# Autodesk Inventor assembly: ExternalMoldAssembly
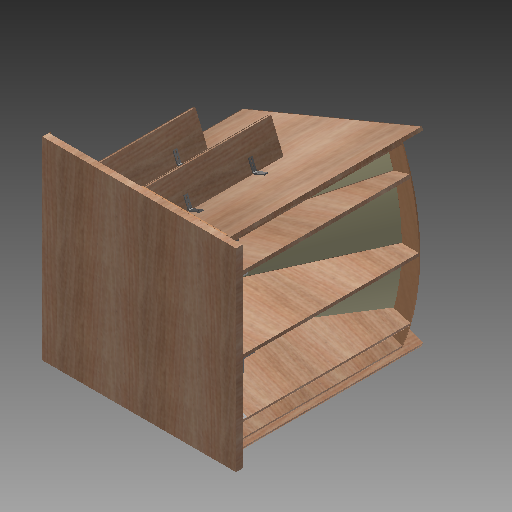
[picture p0: Inventor's stored thumbnail of the model, 512x512]
Saved by Autodesk Inventor 2019 (Build 230136000, 136)
## iProperties
Company: FABLAB Torino
Created: 2019-01-11
Part Number: ExternalMoldAssembly
Document SubType Name: Assembly
Designer: Giancarlo
Project: La Panca - Flower Vase
Mass: 72304.3 g
Surface Area: 89186 cm^2
Volume: 48627 cm^3
Density: 1.48692 g/cm^3
Author: Giancarlo
Title: La Panca - Flower Vase
Subject: Construction MOld
## Documents named in this file (14)
- D:\Giancarlo Bacchio\Documenti\00 - Progetti\30-Inventor\flower vase\ExternalMoldAssembly.iam
- D:\Giancarlo Bacchio\Documenti\00 - Progetti\30-Inventor\flower vase\externalMold_parts\front panel.ipt
- D:\Giancarlo Bacchio\Documenti\00 - Progetti\30-Inventor\flower vase\externalMold_parts\rear panel.ipt
- D:\Giancarlo Bacchio\Documenti\00 - Progetti\30-Inventor\flower vase\externalMold_parts\base1.ipt
- D:\Giancarlo Bacchio\Documenti\00 - Progetti\30-Inventor\flower vase\externalMold_parts\ref1.ipt
- D:\Giancarlo Bacchio\Documenti\00 - Progetti\30-Inventor\flower vase\externalMold_parts\support1.ipt
- D:\Giancarlo Bacchio\Documenti\00 - Progetti\30-Inventor\flower vase\externalMold_parts\frontformer.ipt
- D:\Giancarlo Bacchio\Documenti\00 - Progetti\30-Inventor\flower vase\externalMold_parts\verticalff.ipt
- D:\Giancarlo Bacchio\Documenti\00 - Progetti\30-Inventor\flower vase\externalMold_parts\verticalff1.ipt
- D:\Giancarlo Bacchio\Documenti\00 - Progetti\30-Inventor\flower vase\externalMold_parts\ref3.ipt
- D:\Giancarlo Bacchio\Documenti\00 - Progetti\30-Inventor\flower vase\externalMold_parts\base.ipt
- D:\Giancarlo Bacchio\Documenti\00 - Progetti\30-Inventor\flower vase\externalMold_parts\externalSupportRear1.ipt
- D:\Giancarlo Bacchio\Documenti\00 - Progetti\30-Inventor\flower vase\externalMold_parts\externalSupportRear3.ipt
- D:\Giancarlo Bacchio\Documenti\00 - Progetti\30-Inventor\flower vase\externalMold_parts\JIS G 3350C - 3075     40x40-12.ipt
## Components (53 placed, 13 different names)
1. externalSupportRear3:1 — Flush:19, Flush:20, Mate:86, Mate:88, Mate:90, Mate:92, Mate:94
2. externalSupportRear1:1 — Flush:17, Flush:18
3. externalSupportBase:1 — Flush:19, Flush:20, Mate:76, Mate:78, Mate:80, Mate:82, Mate:84, Mate:106, Flush:26, Mate:120, Mate:125, Flush:27, Mate:126, Mate:128, Mate:130, Mate:132, Mate:133
4. JIS G 3350C - 3075     40x40-12:22 — Mate:133, Mate:135, Flush:31
5. JIS G 3350C - 3075     40x40-12:21 — Mate:132, Mate:137, Flush:32
6. JIS G 3350C - 3075     40x40-12:20 — Mate:128, Mate:136, Flush:33
7. JIS G 3350C - 3075     40x40-12:19 — Mate:126, Mate:127, Flush:28
8. JIS G 3350C - 3075     40x40-12:18 — Mate:116, Mate:117, Mate:118
9. JIS G 3350C - 3075     40x40-12:17 — Mate:114, Mate:115, Mate:124
10. JIS G 3350C - 3075     40x40-12:16 — Mate:112, Mate:113, Mate:123
11. JIS G 3350C - 3075     40x40-12:15 — Mate:110, Mate:111, Mate:119
12. ref1:2 — Mate:106, Mate:107, Flush:26, Mate:108, Mate:109
13. JIS G 3350C - 3075     40x40-12:14 — Mate:103, Mate:104, Mate:109
14. JIS G 3350C - 3075     40x40-12:13 — Mate:102, Mate:105, Mate:108
15. JIS G 3350C - 3075     40x40-12:12 — Mate:99, Mate:100, Mate:101
16. JIS G 3350C - 3075     40x40-12:11 — Mate:88, Mate:89
17. JIS G 3350C - 3075     40x40-12:10 — Mate:94, Mate:95
18. JIS G 3350C - 3075     40x40-12:9 — Mate:96, Mate:97, Mate:98
19. JIS G 3350C - 3075     40x40-12:8 — Mate:92, Mate:93
20. JIS G 3350C - 3075     40x40-12:7 — Mate:90, Mate:91
21. JIS G 3350C - 3075     40x40-12:6 — Mate:86, Mate:87
22. JIS G 3350C - 3075     40x40-12:5 — Mate:84, Mate:85, Flush:25
23. JIS G 3350C - 3075     40x40-12:4 — Mate:82, Mate:83, Flush:24
24. JIS G 3350C - 3075     40x40-12:3 — Mate:80, Mate:81, Flush:23
25. JIS G 3350C - 3075     40x40-12:2 — Mate:78, Mate:79, Flush:22
26. JIS G 3350C - 3075     40x40-12:1 — Mate:76, Mate:77, Flush:21
27. base1:2 — Mate:75, Mate:97, Mate:100, Mate:104, Mate:105
28. base1:3 — Mate:73, Mate:111, Mate:113, Mate:115, Mate:117, Mate:122, Mate:131
29. ref3:1 — Mate:73, Mate:121, Mate:123, Mate:124, Mate:125, Flush:27
30. ref3:2 — Mate:61, Mate:75, Mate:98, Mate:101
31. verticalff1:1 — Mate:81, Flush:23, Mate:91
32. verticalff1:2 — Mate:79, Flush:22, Mate:95
33. verticalff1:3 — Mate:85, Flush:25, Mate:89
34. verticalff1:4 — Flush:17, Flush:18, Mate:77, Flush:21, Mate:93
35. verticalff1:5 — Mate:83, Flush:24, Mate:87
36. frontformer:1 — Flush:10, Flush:11, Flush:12, Mate:17, Flush:13, Mate:19
37. verticalff:1 — Flush:10, Flush:11, Flush:14, Mate:20, Mate:21, Mate:22, Mate:23, Mate:24
38. verticalff:2 — Flush:12, Mate:17
39. verticalff:3 — Flush:13, Mate:19, Mate:25, Mate:26, Mate:27, Mate:28, Mate:29, Mate:30, Mate:31, Mate:32, Mate:33, Mate:34, Mate:35, Mate:36, Mate:37, Mate:38, Mate:39, Mate:40
40. frontformer:2 — Flush:14, Mate:20, Mate:21, Mate:22
41. frontformer:3 — Mate:23, Mate:24, Mate:25
42. frontformer:4 — Mate:26, Mate:27, Mate:28
43. frontformer:5 — Mate:29, Mate:30, Mate:31
44. frontformer:6 — Mate:32, Mate:33, Mate:34
45. frontformer:7 — Mate:38, Mate:39, Mate:40
46. frontformer:8 — Mate:35, Mate:36, Mate:37
47. ref1:1 — Mate:12, Mate:118, Mate:119
48. support1:1 — Mate:112, Mate:114, Mate:120, Mate:121, Mate:122, Mate:135, Flush:31
49. support1:2 — Mate:12, Mate:110, Mate:116, Mate:127, Mate:130, Mate:131, Flush:28
50. support1:3 — Mate:102, Mate:103, Mate:107, Mate:136, Flush:33
51. support1:4 — Mate:61, Mate:96, Mate:99, Mate:137, Flush:32
52. front panel:1
53. rear panel:1
## Relationships (107: Mate 87, Flush 20)
- Mate:12: ref1:1 ↔ support1:2
- Flush:10: frontformer:1 ↔ verticalff:1
- Flush:11: frontformer:1 ↔ verticalff:1
- Flush:12: frontformer:1 ↔ verticalff:2
- Mate:17: frontformer:1 ↔ verticalff:2
- Flush:13: frontformer:1 ↔ verticalff:3
- Mate:19: frontformer:1 ↔ verticalff:3
- Flush:14: verticalff:1 ↔ frontformer:2
- Mate:20: verticalff:1 ↔ frontformer:2
- Mate:21: verticalff:1 ↔ frontformer:2
- Mate:22: verticalff:1 ↔ frontformer:2
- Mate:23: verticalff:1 ↔ frontformer:3
- Mate:24: verticalff:1 ↔ frontformer:3
- Mate:25: verticalff:3 ↔ frontformer:3
- Mate:26: verticalff:3 ↔ frontformer:4
- Mate:27: verticalff:3 ↔ frontformer:4
- Mate:28: verticalff:3 ↔ frontformer:4
- Mate:29: verticalff:3 ↔ frontformer:5
- Mate:30: verticalff:3 ↔ frontformer:5
- Mate:31: verticalff:3 ↔ frontformer:5
- Mate:32: verticalff:3 ↔ frontformer:6
- Mate:33: verticalff:3 ↔ frontformer:6
- Mate:34: verticalff:3 ↔ frontformer:6
- Mate:35: verticalff:3 ↔ frontformer:8
- Mate:36: verticalff:3 ↔ frontformer:8
- Mate:37: verticalff:3 ↔ frontformer:8
- Mate:38: verticalff:3 ↔ frontformer:7
- Mate:39: verticalff:3 ↔ frontformer:7
- Mate:40: verticalff:3 ↔ frontformer:7
- Mate:61: ref3:2 ↔ support1:4
- Mate:73: base1:3 ↔ ref3:1
- Mate:75: base1:2 ↔ ref3:2
- Flush:17: externalSupportRear1:1 ↔ verticalff1:4
- Flush:18: externalSupportRear1:1 ↔ verticalff1:4
- Flush:19: externalSupportRear3:1 ↔ externalSupportBase:1
- Flush:20 (4 mm): externalSupportRear3:1 ↔ externalSupportBase:1
- Mate:76: externalSupportBase:1 ↔ JIS G 3350C - 3075     40x40-12:1
- Mate:77: JIS G 3350C - 3075     40x40-12:1 ↔ verticalff1:4
- Flush:21: JIS G 3350C - 3075     40x40-12:1 ↔ verticalff1:4
- Mate:78: externalSupportBase:1 ↔ JIS G 3350C - 3075     40x40-12:2
- Mate:79: JIS G 3350C - 3075     40x40-12:2 ↔ verticalff1:2
- Flush:22: JIS G 3350C - 3075     40x40-12:2 ↔ verticalff1:2
- Mate:80: externalSupportBase:1 ↔ JIS G 3350C - 3075     40x40-12:3
- Mate:81: JIS G 3350C - 3075     40x40-12:3 ↔ verticalff1:1
- Flush:23: JIS G 3350C - 3075     40x40-12:3 ↔ verticalff1:1
- Mate:82: externalSupportBase:1 ↔ JIS G 3350C - 3075     40x40-12:4
- Mate:83: JIS G 3350C - 3075     40x40-12:4 ↔ verticalff1:5
- Flush:24: JIS G 3350C - 3075     40x40-12:4 ↔ verticalff1:5
- Mate:84: externalSupportBase:1 ↔ JIS G 3350C - 3075     40x40-12:5
- Mate:85: JIS G 3350C - 3075     40x40-12:5 ↔ verticalff1:3
- Flush:25: JIS G 3350C - 3075     40x40-12:5 ↔ verticalff1:3
- Mate:86: externalSupportRear3:1 ↔ JIS G 3350C - 3075     40x40-12:6
- Mate:87: JIS G 3350C - 3075     40x40-12:6 ↔ verticalff1:5
- Mate:88: externalSupportRear3:1 ↔ JIS G 3350C - 3075     40x40-12:11
- Mate:89: JIS G 3350C - 3075     40x40-12:11 ↔ verticalff1:3
- Mate:90: externalSupportRear3:1 ↔ JIS G 3350C - 3075     40x40-12:7
- Mate:91: JIS G 3350C - 3075     40x40-12:7 ↔ verticalff1:1
- Mate:92: externalSupportRear3:1 ↔ JIS G 3350C - 3075     40x40-12:8
- Mate:93: JIS G 3350C - 3075     40x40-12:8 ↔ verticalff1:4
- Mate:94: externalSupportRear3:1 ↔ JIS G 3350C - 3075     40x40-12:10
- Mate:95: JIS G 3350C - 3075     40x40-12:10 ↔ verticalff1:2
- Mate:96: JIS G 3350C - 3075     40x40-12:9 ↔ support1:4
- Mate:97: JIS G 3350C - 3075     40x40-12:9 ↔ base1:2
- Mate:98 (100 mm): JIS G 3350C - 3075     40x40-12:9 ↔ ref3:2
- Mate:99: JIS G 3350C - 3075     40x40-12:12 ↔ support1:4
- Mate:100: JIS G 3350C - 3075     40x40-12:12 ↔ base1:2
- Mate:101 (300 mm): JIS G 3350C - 3075     40x40-12:12 ↔ ref3:2
- Mate:102: JIS G 3350C - 3075     40x40-12:13 ↔ support1:3
- Mate:103: JIS G 3350C - 3075     40x40-12:14 ↔ support1:3
- Mate:104: JIS G 3350C - 3075     40x40-12:14 ↔ base1:2
- Mate:105: JIS G 3350C - 3075     40x40-12:13 ↔ base1:2
- Mate:106: externalSupportBase:1 ↔ ref1:2
- Mate:107: ref1:2 ↔ support1:3
- Flush:26: externalSupportBase:1 ↔ ref1:2
- Mate:108 (100 mm): ref1:2 ↔ JIS G 3350C - 3075     40x40-12:13
- Mate:109 (300 mm): ref1:2 ↔ JIS G 3350C - 3075     40x40-12:14
- Mate:110: JIS G 3350C - 3075     40x40-12:15 ↔ support1:2
- Mate:111: JIS G 3350C - 3075     40x40-12:15 ↔ base1:3
- Mate:112: JIS G 3350C - 3075     40x40-12:16 ↔ support1:1
- Mate:113: JIS G 3350C - 3075     40x40-12:16 ↔ base1:3
- Mate:114: JIS G 3350C - 3075     40x40-12:17 ↔ support1:1
- Mate:115: JIS G 3350C - 3075     40x40-12:17 ↔ base1:3
- Mate:116: JIS G 3350C - 3075     40x40-12:18 ↔ support1:2
- Mate:117: JIS G 3350C - 3075     40x40-12:18 ↔ base1:3
- Mate:118 (100 mm): JIS G 3350C - 3075     40x40-12:18 ↔ ref1:1
- Mate:119 (300 mm): JIS G 3350C - 3075     40x40-12:15 ↔ ref1:1
- Mate:120: externalSupportBase:1 ↔ support1:1
- Mate:121: ref3:1 ↔ support1:1
- Mate:122: base1:3 ↔ support1:1
- Mate:123 (100 mm): JIS G 3350C - 3075     40x40-12:16 ↔ ref3:1
- Mate:124 (300 mm): JIS G 3350C - 3075     40x40-12:17 ↔ ref3:1
- Mate:125: externalSupportBase:1 ↔ ref3:1
- Flush:27: externalSupportBase:1 ↔ ref3:1
- Mate:126: externalSupportBase:1 ↔ JIS G 3350C - 3075     40x40-12:19
- Mate:127: JIS G 3350C - 3075     40x40-12:19 ↔ support1:2
- Mate:128: externalSupportBase:1 ↔ JIS G 3350C - 3075     40x40-12:20
- Mate:130: externalSupportBase:1 ↔ support1:2
- Mate:131: base1:3 ↔ support1:2
- Flush:28 (10 mm): JIS G 3350C - 3075     40x40-12:19 ↔ support1:2
- Mate:132: externalSupportBase:1 ↔ JIS G 3350C - 3075     40x40-12:21
- Mate:133: externalSupportBase:1 ↔ JIS G 3350C - 3075     40x40-12:22
- Mate:135: JIS G 3350C - 3075     40x40-12:22 ↔ support1:1
- Flush:31 (10 mm): JIS G 3350C - 3075     40x40-12:22 ↔ support1:1
- Mate:136: JIS G 3350C - 3075     40x40-12:20 ↔ support1:3
- Mate:137: JIS G 3350C - 3075     40x40-12:21 ↔ support1:4
- Flush:32 (10 mm): JIS G 3350C - 3075     40x40-12:21 ↔ support1:4
- Flush:33 (10 mm): JIS G 3350C - 3075     40x40-12:20 ↔ support1:3
